# Autodesk Inventor assembly: Link2
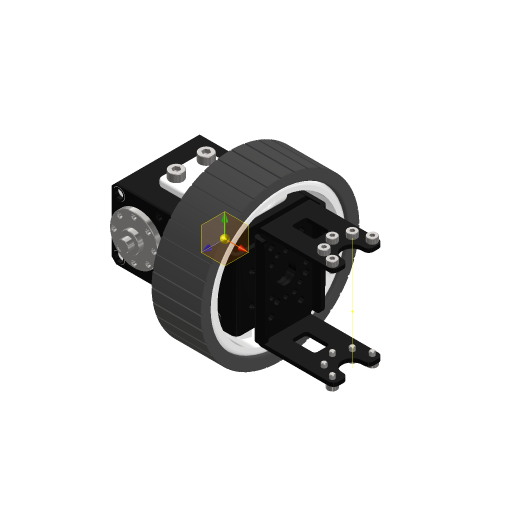
[picture p0: Inventor's stored thumbnail of the model, 512x512]
Saved by Autodesk Inventor 2024 (Build 280153000, 153)
## iProperties
Created: 2022-11-03
Part Number: Link2
Document SubType Name: Assembly
Designer: doore
Mass: 123.815 g
Surface Area: 411.684 cm^2
Volume: 81.3149 cm^3
Density: 1.52266 g/cm^3
Author: doore
## Documents named in this file (8)
- C:\Users\Bong\project\snake_RL\matlab\meshes\Inventor_Reallign\linkA\LinkA.iam
- C:\Users\Bong\project\snake_RL\matlab\meshes\Inventor_Reallign\linkA\xm430.ipt
- C:\Users\Bong\project\snake_RL\matlab\meshes\Inventor_Reallign\linkA\solid_circular_frame.ipt
- C:\Users\Bong\Documents\Inventor\Content Center Files\R2024\ko-KR\BS EN ISO 4762\BS EN ISO 4762 - M3 x 5(1).ipt
- C:\Users\Bong\project\snake_RL\matlab\meshes\Inventor_Reallign\linkA\xm430_frame.ipt
- C:\Users\Bong\project\snake_RL\matlab\meshes\Inventor_Reallign\linkA\xm430_hinge.ipt
- C:\Users\Bong\Documents\Inventor\Content Center Files\R2024\ko-KR\BS 4168(1)\BS 4168 - M2 x 3(1).ipt
- C:\Users\Bong\project\snake_RL\matlab\meshes\Inventor_Reallign\linkA\rubber.ipt
## Components (19 placed, 7 different names)
1. xm430:1 — 강체:1, 강체:6, 플러쉬:1, 플러쉬:2
2. solid_circular_frame:1 — 강체:1, 강체:2, 강체:3, 강체:4, 강체:5, 강체:18
3. BS EN ISO 4762 : 부품 1 6각 소켓 머리 캡 나사 - 미터 M3 x 5:1 — 강체:2
4. BS EN ISO 4762 : 부품 1 6각 소켓 머리 캡 나사 - 미터 M3 x 5:2 — 강체:3
5. BS EN ISO 4762 : 부품 1 6각 소켓 머리 캡 나사 - 미터 M3 x 5:3 — 강체:4
6. BS EN ISO 4762 : 부품 1 6각 소켓 머리 캡 나사 - 미터 M3 x 5:4 — 강체:5
7. xm430_frame:1 — 강체:6, 강체:7
8. xm430_hinge:1 — 강체:7, 강체:8, 강체:9, 강체:10, 강체:11, 강체:12, 강체:13, 강체:14, 강체:15, 강체:16, 강체:17, 메이트:1
9. BS 4168 : 부품 1 6각 소켓 머리 캡 나사 - 미터 M2 x 3:1 — 강체:8
10. BS 4168 : 부품 1 6각 소켓 머리 캡 나사 - 미터 M2 x 3:2 — 강체:9
11. BS 4168 : 부품 1 6각 소켓 머리 캡 나사 - 미터 M2 x 3:3 — 강체:10
12. BS 4168 : 부품 1 6각 소켓 머리 캡 나사 - 미터 M2 x 3:4 — 강체:11
13. BS 4168 : 부품 1 6각 소켓 머리 캡 나사 - 미터 M2 x 3:5 — 강체:12
14. BS 4168 : 부품 1 6각 소켓 머리 캡 나사 - 미터 M2 x 3:6 — 강체:13
15. BS 4168 : 부품 1 6각 소켓 머리 캡 나사 - 미터 M2 x 3:7 — 강체:14
16. BS 4168 : 부품 1 6각 소켓 머리 캡 나사 - 미터 M2 x 3:8 — 강체:15
17. BS 4168 : 부품 1 6각 소켓 머리 캡 나사 - 미터 M2 x 3:9 — 강체:16
18. BS 4168 : 부품 1 6각 소켓 머리 캡 나사 - 미터 M2 x 3:10 — 강체:17
19. rubber:1 — 강체:18
## Relationships (22: WeldJoint 18, Mate 2, Flush 2)
- 강체:1 [WeldJoint]: xm430:1 ↔ solid_circular_frame:1
- 강체:2 [WeldJoint]: solid_circular_frame:1 ↔ BS EN ISO 4762 : 부품 1 6각 소켓 머리 캡 나사 - 미터 M3 x 5:1
- 강체:3 [WeldJoint]: solid_circular_frame:1 ↔ BS EN ISO 4762 : 부품 1 6각 소켓 머리 캡 나사 - 미터 M3 x 5:2
- 강체:4 [WeldJoint]: solid_circular_frame:1 ↔ BS EN ISO 4762 : 부품 1 6각 소켓 머리 캡 나사 - 미터 M3 x 5:3
- 강체:5 [WeldJoint]: solid_circular_frame:1 ↔ BS EN ISO 4762 : 부품 1 6각 소켓 머리 캡 나사 - 미터 M3 x 5:4
- 강체:6 [WeldJoint]: xm430:1 ↔ xm430_frame:1
- 강체:7 [WeldJoint]: xm430_frame:1 ↔ xm430_hinge:1
- 강체:8 [WeldJoint]: xm430_hinge:1 ↔ BS 4168 : 부품 1 6각 소켓 머리 캡 나사 - 미터 M2 x 3:1
- 강체:9 [WeldJoint]: xm430_hinge:1 ↔ BS 4168 : 부품 1 6각 소켓 머리 캡 나사 - 미터 M2 x 3:2
- 강체:10 [WeldJoint]: xm430_hinge:1 ↔ BS 4168 : 부품 1 6각 소켓 머리 캡 나사 - 미터 M2 x 3:3
- 강체:11 [WeldJoint]: xm430_hinge:1 ↔ BS 4168 : 부품 1 6각 소켓 머리 캡 나사 - 미터 M2 x 3:4
- 강체:12 [WeldJoint]: xm430_hinge:1 ↔ BS 4168 : 부품 1 6각 소켓 머리 캡 나사 - 미터 M2 x 3:5
- 강체:13 [WeldJoint]: xm430_hinge:1 ↔ BS 4168 : 부품 1 6각 소켓 머리 캡 나사 - 미터 M2 x 3:6
- 강체:14 [WeldJoint]: xm430_hinge:1 ↔ BS 4168 : 부품 1 6각 소켓 머리 캡 나사 - 미터 M2 x 3:7
- 강체:15 [WeldJoint]: xm430_hinge:1 ↔ BS 4168 : 부품 1 6각 소켓 머리 캡 나사 - 미터 M2 x 3:8
- 강체:16 [WeldJoint]: xm430_hinge:1 ↔ BS 4168 : 부품 1 6각 소켓 머리 캡 나사 - 미터 M2 x 3:9
- 강체:17 [WeldJoint]: xm430_hinge:1 ↔ BS 4168 : 부품 1 6각 소켓 머리 캡 나사 - 미터 M2 x 3:10
- 강체:18 [WeldJoint]: solid_circular_frame:1 ↔ rubber:1
- 메이트:1 [Mate]: xm430_hinge:1
- 메이트:2 [Mate]
- 플러쉬:1 [Flush]: xm430:1
- 플러쉬:2 [Flush]: xm430:1
